# Autodesk Inventor assembly: 2A.01.01.01.IM.FlapAssembly
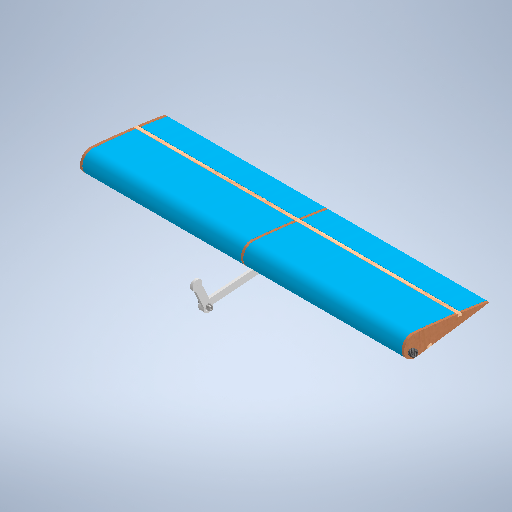
[picture p0: Inventor's stored thumbnail of the model, 512x512]
Saved by Autodesk Inventor 2025.2 (Build 292293000, 293)
## iProperties
Created: 2025-01-27
Part Number: 2A.01.01.01.IM.FlapAssembly
Document SubType Name: Assembly
Designer: Imist
Author: Imist
## Documents named in this file (14)
- C:\Users\Imist\OneDrive - University of Bristol\Year 2\AVDASI 2\Team\Final CAD\2A.01.01.01.IM.FlapAssembly.iam
- C:\Users\Imist\OneDrive - University of Bristol\Year 2\AVDASI 2\Team\Final CAD\2P.03.01.01.IM.FlapBody.ipt
- C:\Users\Imist\OneDrive - University of Bristol\Year 2\AVDASI 2\Team\Final CAD\2P.03.01.04.IM.FlapSpar.ipt
- C:\Users\Imist\OneDrive - University of Bristol\Year 2\AVDASI 2\Team\Final CAD\2P.03.01.05.IM.FlapCutFill.ipt
- C:\Users\Imist\OneDrive - University of Bristol\Year 2\AVDASI 2\Team\Final CAD\2P.03.01.07.JW.FlapRibMid.ipt
- C:\Users\Imist\OneDrive - University of Bristol\Year 2\AVDASI 2\Team\Final CAD\2P.03.01.09.IM.FlapRibEnd.ipt
- C:\Users\Imist\OneDrive - University of Bristol\Year 2\AVDASI 2\Team\Final CAD\2P.03.01.15.ZW.FlapCoupler.ipt
- C:\Users\Imist\OneDrive - University of Bristol\Year 2\AVDASI 2\Team\Final CAD\2P.03.01.16.ZW.FlapCrank.ipt
- C:\Users\Imist\OneDrive - University of Bristol\Year 2\AVDASI 2\Team\Final CAD\2P.03.01.11.IM.FlapBottSpanBeam.ipt
- C:\Users\Imist\OneDrive - University of Bristol\Year 2\AVDASI 2\Team\Final CAD\2P.03.01.12.IM.FlapTopSpanBeam.ipt
- C:\Users\Imist\OneDrive\Documents\Inventor\Content Center Files\R2025\en-US\ISO 7092\ISO 7092 - ST 3 - 140 HV.ipt
- C:\Users\Imist\OneDrive\Documents\Inventor\Content Center Files\R2025\en-US\ISO 4032(2)\ISO 4032 - M3 - ISO.ipt
- C:\Users\Imist\OneDrive\Documents\Inventor\Content Center Files\R2025\en-US\AS 1420\AS 1420 - 1973 - M3 x 12.ipt
- C:\Users\Imist\OneDrive - University of Bristol\Year 2\AVDASI 2\Team\Final CAD\2P.03.01.00.01.IM.Bearing3x7x3.ipt
## Components (26 placed, 13 different names)
1. 2P.03.01.01.IM.FlapBody:1 — Rigid:1, Rigid:4, Rigid:5
2. 2P.03.01.04.IM.FlapSpar:1 — Mate:1, Mate:2, Mate:3, Mate:4, Rigid:19
3. 2P.03.01.05.IM.FlapCutFill:1 — Rigid:1
4. 2P.03.01.07.JW.FlapRibMid:1 — Rigid:3, Rigid:4, Rigid:15, Rigid:19
5. 2P.03.01.09.IM.FlapRibEnd:1 — Rigid:6, Rigid:7
6. 2P.03.01.15.ZW.FlapCoupler:1 — Rigid:16, Rigid:17
7. 2P.03.01.16.ZW.FlapCrank:1 — Rigid:18
8. 2P.03.01.01.IM.FlapBody:2 — Rigid:3, Rigid:6
9. 2P.03.01.05.IM.FlapCutFill:2
10. 2P.03.01.09.IM.FlapRibEnd:2 — Rigid:5, Rigid:8
11. 2P.03.01.11.IM.FlapBottSpanBeam:1 — Rigid:8
12. 2P.03.01.12.IM.FlapTopSpanBeam:1 — Rigid:7
13. ISO 7092 ST 3 - 140 HV:1 — Rotational:16, Rotational:19
14. ISO 7092 ST 3 - 140 HV:2 — Rotational:12, Rotational:17
15. ISO 7092 ST 3 - 140 HV:3 — Rotational:14, Rotational:18
16. ISO 7092 ST 3 - 140 HV:4 — Rotational:20, Rotational:21
17. ISO 7092 ST 3 - 140 HV:5 — Rotational:11, Rotational:23
18. ISO 7092 ST 3 - 140 HV:6 — Rotational:13, Rotational:22
19. ISO 4032 M3:1 — Rotational:11
20. AS 1420 - Metric M3 x 12:1 — Rotational:12
21. AS 1420 - Metric M3 x 12:2 — Rotational:13
22. ISO 4032 M3:2 — Rotational:14
23. 2P.03.01.00.01.IM.Bearing3x7x3:1 — Rigid:15, Rotational:16, Rotational:18
24. 2P.03.01.00.01.IM.Bearing3x7x3:2 — Rigid:16, Rotational:17, Rotational:19
25. 2P.03.01.00.01.IM.Bearing3x7x3:3 — Rigid:18, Rotational:21, Rotational:22
26. 2P.03.01.00.01.IM.Bearing3x7x3:4 — Rigid:17, Rotational:20, Rotational:23
## Relationships (29: WeldJoint 13, RevoluteJoint 12, Mate 4)
- Rigid:1 [WeldJoint]: 2P.03.01.01.IM.FlapBody:1 ↔ 2P.03.01.05.IM.FlapCutFill:1
- [WeldJoint]: 2P.03.01.01.IM.FlapBody:2 ↔ 2P.03.01.05.IM.FlapCutFill:2
- Rigid:3 [WeldJoint]: 2P.03.01.07.JW.FlapRibMid:1 ↔ 2P.03.01.01.IM.FlapBody:2
- Rigid:4 [WeldJoint]: 2P.03.01.01.IM.FlapBody:1 ↔ 2P.03.01.07.JW.FlapRibMid:1
- Rigid:5 [WeldJoint]: 2P.03.01.01.IM.FlapBody:1 ↔ 2P.03.01.09.IM.FlapRibEnd:2
- Rigid:6 [WeldJoint]: 2P.03.01.09.IM.FlapRibEnd:1 ↔ 2P.03.01.01.IM.FlapBody:2
- Rigid:7 [WeldJoint]: 2P.03.01.09.IM.FlapRibEnd:1 ↔ 2P.03.01.12.IM.FlapTopSpanBeam:1
- Rigid:8 [WeldJoint]: 2P.03.01.09.IM.FlapRibEnd:2 ↔ 2P.03.01.11.IM.FlapBottSpanBeam:1
- Rotational:11 [RevoluteJoint]: ISO 7092 ST 3 - 140 HV:5 ↔ ISO 4032 M3:1
- Rotational:12 [RevoluteJoint]: ISO 7092 ST 3 - 140 HV:2 ↔ AS 1420 - Metric M3 x 12:1
- Rotational:13 [RevoluteJoint]: ISO 7092 ST 3 - 140 HV:6 ↔ AS 1420 - Metric M3 x 12:2
- Rotational:14 [RevoluteJoint] (2.4 mm): ISO 7092 ST 3 - 140 HV:3 ↔ ISO 4032 M3:2
- Rigid:15 [WeldJoint]: 2P.03.01.07.JW.FlapRibMid:1 ↔ 2P.03.01.00.01.IM.Bearing3x7x3:1
- Rigid:16 [WeldJoint]: 2P.03.01.15.ZW.FlapCoupler:1 ↔ 2P.03.01.00.01.IM.Bearing3x7x3:2
- Rigid:17 [WeldJoint]: 2P.03.01.15.ZW.FlapCoupler:1 ↔ 2P.03.01.00.01.IM.Bearing3x7x3:4
- Rigid:18 [WeldJoint]: 2P.03.01.16.ZW.FlapCrank:1 ↔ 2P.03.01.00.01.IM.Bearing3x7x3:3
- Rotational:16 [RevoluteJoint] (0.5 mm): ISO 7092 ST 3 - 140 HV:1 ↔ 2P.03.01.00.01.IM.Bearing3x7x3:1
- Rotational:17 [RevoluteJoint]: ISO 7092 ST 3 - 140 HV:2 ↔ 2P.03.01.00.01.IM.Bearing3x7x3:2
- Rotational:18 [RevoluteJoint]: ISO 7092 ST 3 - 140 HV:3 ↔ 2P.03.01.00.01.IM.Bearing3x7x3:1
- Rotational:19 [RevoluteJoint]: ISO 7092 ST 3 - 140 HV:1 ↔ 2P.03.01.00.01.IM.Bearing3x7x3:2
- Rotational:20 [RevoluteJoint] (0.5 mm): ISO 7092 ST 3 - 140 HV:4 ↔ 2P.03.01.00.01.IM.Bearing3x7x3:4
- Rotational:21 [RevoluteJoint]: ISO 7092 ST 3 - 140 HV:4 ↔ 2P.03.01.00.01.IM.Bearing3x7x3:3
- Rotational:22 [RevoluteJoint]: ISO 7092 ST 3 - 140 HV:6 ↔ 2P.03.01.00.01.IM.Bearing3x7x3:3
- Rotational:23 [RevoluteJoint]: ISO 7092 ST 3 - 140 HV:5 ↔ 2P.03.01.00.01.IM.Bearing3x7x3:4
- Mate:1: 2P.03.01.04.IM.FlapSpar:1
- Mate:2: 2P.03.01.04.IM.FlapSpar:1
- Mate:3: 2P.03.01.04.IM.FlapSpar:1
- Mate:4: 2P.03.01.04.IM.FlapSpar:1
- Rigid:19 [WeldJoint] (-1.5 mm): 2P.03.01.04.IM.FlapSpar:1 ↔ 2P.03.01.07.JW.FlapRibMid:1
## Named parameters: d1_d0 = 0 mm
